# Autodesk Inventor assembly: MainDrone
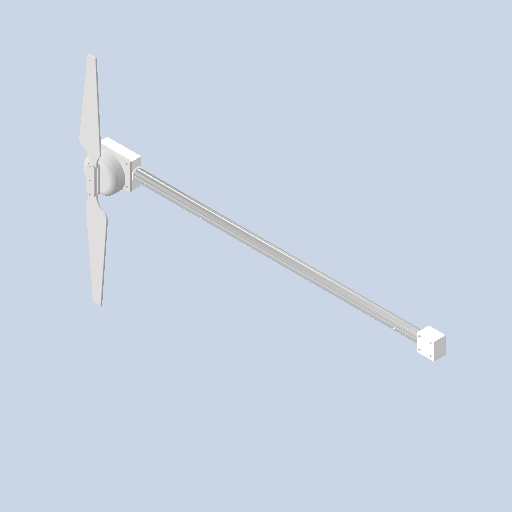
[picture p0: Inventor's stored thumbnail of the model, 512x512]
Saved by Autodesk Inventor 2022.1 (Build 261234020, 234B)
## iProperties
Created: 2021-11-14
Part Number: MainDrone
Document SubType Name: Assembly
Designer: Alexander
Author: Alexander
## Documents named in this file (11)
- C:\Users\Alexander\Desktop\upload\Drone\3D models\Arm.iam
- C:\Users\Alexander\Desktop\upload\Drone\3D models\BodyTube.ipt
- C:\Users\Alexander\Desktop\upload\Drone\3D models\MotorHolderv2.ipt
- C:\Users\Alexander\Desktop\upload\Drone\3D models\RodConnector.ipt
- C:\Users\Alexander\Desktop\upload\Drone\3D models\Motor\FullMotor.iam
- C:\Users\Alexander\Desktop\Drone\inventor\MainDrone\AIP\FEA\dsefciag0.fins
- C:\Users\Alexander\Desktop\Drone\inventor\MainDrone\AIP\FEA\dsefciag0.fsat
- C:\Users\Alexander\Desktop\Drone\inventor\MainDrone\AIP\FEA\dsefciag0.ftes
- C:\Users\Alexander\Desktop\Drone\inventor\MainDrone\AIP\FEA\dsefciag0.fwiz
- C:\Users\Alexander\Desktop\Drone\inventor\MainDrone\AIP\FEA\dsefciag1.fmsh
- C:\Users\Alexander\Desktop\Drone\inventor\MainDrone\AIP\FEA\dsefciag2.fres
## Components (4 placed, 4 different names)
1. BodyTube:1 — Rigid:1, Rigid:2
2. MotorHolderv2:1 — Rigid:1, Angle:1, Mate:1, Mate:2, Mate:3
3. RodConnector:1 — Rigid:2, Angle:1
4. FullMotor:1 [sub-assembly] — Mate:1, Mate:2, Mate:3
## Relationships (6: Mate 3, WeldJoint 2, Angle 1)
- Rigid:1 [WeldJoint]: BodyTube:1 ↔ MotorHolderv2:1
- Rigid:2 [WeldJoint]: BodyTube:1 ↔ RodConnector:1
- Angle:1 (0 deg): MotorHolderv2:1 ↔ RodConnector:1
- Mate:1: MotorHolderv2:1 ↔ FullMotor:1
- Mate:2: MotorHolderv2:1 ↔ FullMotor:1
- Mate:3: MotorHolderv2:1 ↔ FullMotor:1
## Named parameters: sa_0 = 4000
note: some values were not read from the file. Shown as the stored number, unit unknown: "sa_0".
